# Autodesk Inventor assembly: ArmadoNewtonCart
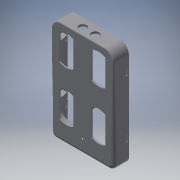
[picture p0: Inventor's stored thumbnail of the model, 180x180]
Saved by Autodesk Inventor 2018 (Build 220112000, 112)
## iProperties
Created: 2020-10-10
Part Number: ArmadoNewtonCart
Document SubType Name: Assembly
Designer: peter
Author: peter
## Documents named in this file (3)
- C:\Users\peter\Documents\GitHub\Newton-Cart2\3D Platform design\ArmadoNewtonCart.iam
- C:\Users\peter\Documents\GitHub\Newton-Cart2\3D Platform design\Carcasa1.ipt
- C:\Users\peter\Documents\GitHub\Newton-Cart2\3D Platform design\garracomp3.ipt
## Components (5 placed, 2 different names)
1. Carcasa1:1 — Mate:1, Mate:2, Mate:3, Mate:4, Mate:5, Mate:6, Mate:7, Mate:8, Mate:9, Mate:10, Mate:11, Mate:12
2. garracomp3:1 — Mate:1, Mate:2, Mate:3
3. garracomp3:2 — Mate:6, Mate:7, Mate:11
4. garracomp3:3 — Mate:8, Mate:9, Mate:10
5. garracomp3:4 — Mate:4, Mate:5, Mate:12
## Relationships (12: Mate 12)
- Mate:1: Carcasa1:1 ↔ garracomp3:1
- Mate:2: Carcasa1:1 ↔ garracomp3:1
- Mate:3: Carcasa1:1 ↔ garracomp3:1
- Mate:4: Carcasa1:1 ↔ garracomp3:4
- Mate:5: Carcasa1:1 ↔ garracomp3:4
- Mate:6: Carcasa1:1 ↔ garracomp3:2
- Mate:7: Carcasa1:1 ↔ garracomp3:2
- Mate:8: Carcasa1:1 ↔ garracomp3:3
- Mate:9: Carcasa1:1 ↔ garracomp3:3
- Mate:10: Carcasa1:1 ↔ garracomp3:3
- Mate:11: Carcasa1:1 ↔ garracomp3:2
- Mate:12: Carcasa1:1 ↔ garracomp3:4
